# Autodesk Inventor assembly: richtigPlaneten
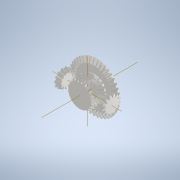
[picture p0: Inventor's stored thumbnail of the model, 180x180]
Saved by Autodesk Inventor 2021 (Build 250183000, 183)
## iProperties
Created: 2021-01-28
Part Number: richtigPlaneten
Document SubType Name: Assembly
Designer: LETPJG
Author: LETPJG
## Documents named in this file (5)
- C:\Users\LETPJG\Documents\Vault\Gruppen\Gruppe 2\Entwurf\Amphibienfahrzeug\richtigPlaneten.iam
- C:\Users\LETPJG\Documents\Vault\Gruppen\Gruppe 2\Entwurf\Amphibienfahrzeug\Planeten\Konstruktions-Assistent\Kegelräder1.iam
- C:\Users\LETPJG\Documents\Vault\Gruppen\Gruppe 2\Entwurf\Amphibienfahrzeug\Planeten\Konstruktions-Assistent\Kegelräder2.iam
- C:\Users\LETPJG\Documents\Vault\Gruppen\Gruppe 2\Entwurf\Amphibienfahrzeug\Planeten\Konstruktions-Assistent\Kegelräder15.iam
- C:\Users\LETPJG\Documents\Vault\Gruppen\Gruppe 2\Entwurf\Amphibienfahrzeug\Planeten\Konstruktions-Assistent\Kegelräder15_MIR.iam
## Components (4 placed, 2 different names)
1. Kegelräder:1 [sub-assembly] — Passend:1, Passend:2, Passend:3, Passend:4, Passend:6
2. Kegelräder:2 [sub-assembly] — Passend:1, Passend:2, Winkel:1
3. Kegelräder:3 [sub-assembly] — Passend:3, Winkel:1, Passend:4, Passend:5
4. Kegelräder15_MIR:1 [sub-assembly] — Passend:5, Passend:6
## Relationships (7: Mate 6, Angle 1)
- Passend:1 [Mate]: Kegelräder:1 ↔ Kegelräder:2
- Passend:2 [Mate]: Kegelräder:1 ↔ Kegelräder:2
- Passend:3 [Mate]: Kegelräder:1 ↔ Kegelräder:3
- Winkel:1 [Angle] (90 deg): Kegelräder:2 ↔ Kegelräder:3
- Passend:4 [Mate]: Kegelräder:1 ↔ Kegelräder:3
- Passend:5 [Mate]: Kegelräder:3 ↔ Kegelräder15_MIR:1
- Passend:6 [Mate] (90 mm): Kegelräder:1 ↔ Kegelräder15_MIR:1
